# Autodesk Inventor assembly: Tracker V4
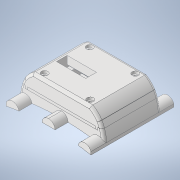
[picture p0: Inventor's stored thumbnail of the model, 180x180]
Saved by Autodesk Inventor 2020 (Build 240168000, 168)
## iProperties
Created: 2019-07-17
Part Number: Tracker V4
Document SubType Name: Assembly
Designer: tyrre
Author: tyrre
## Documents named in this file (3)
- C:\Users\tyrre\OneDrive\Desktop\University - Ryan\Work\Work - 2019\Inventor Files\Tracker V4\Tracker V4.iam
- C:\Users\tyrre\OneDrive\Desktop\University - Ryan\Work\Work - 2019\Inventor Files\Tracker V4\Enclosure-Top.ipt
- C:\Users\tyrre\OneDrive\Desktop\University - Ryan\Work\Work - 2019\Inventor Files\Tracker V4\Enclosure-Base.ipt
## Components (2 placed, 2 different names)
1. Enclosure-Base:1 — Mate:1, Mate:2, Mate:3
2. Enclosure-Top:1 — Mate:1, Mate:2, Mate:3
## Relationships (3: Mate 3)
- Mate:1: Enclosure-Base:1 ↔ Enclosure-Top:1
- Mate:2: Enclosure-Base:1 ↔ Enclosure-Top:1
- Mate:3: Enclosure-Base:1 ↔ Enclosure-Top:1
